# Autodesk Inventor assembly: 組合1
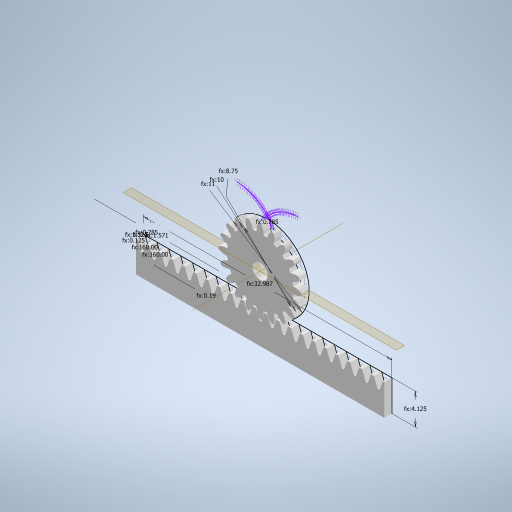
[picture p0: Inventor's stored thumbnail of the model, 512x512]
Saved by Autodesk Inventor 2024 (Build 280153000, 153)
## iProperties
Created: 2024-04-20
Part Number: 組合1
Document SubType Name: Assembly
Designer: rumse
Author: rumse
## Documents named in this file (3)
- C:\文件\機電系統實驗\Electromechanical-System-Principles\抬升機構.iam
- C:\文件\機電系統實驗\Electromechanical-System-Principles\齒條.ipt
- C:\文件\機電系統實驗\Electromechanical-System-Principles\齒輪.ipt
## Components (2 placed, 2 different names)
1. 齒輪:1 — 貼合:1, 相切:1, 貼合:2, 貼合:3, 齊平:1, 貼合:4, 旋轉/轉換:1
2. 齒條:1 — 相切:1, 貼合:2, 齊平:1, 貼合:4, 旋轉/轉換:1, 角度:1
## Relationships (8: Mate 4, Tangent 1, Flush 1, RelateRotateTranslate 1, Angle 1)
- 貼合:1 [Mate]: 齒輪:1
- 相切:1 [Tangent]: 齒輪:1 ↔ 齒條:1
- 貼合:2 [Mate]: 齒輪:1 ↔ 齒條:1
- 貼合:3 [Mate]: 齒輪:1
- 齊平:1 [Flush]: 齒輪:1 ↔ 齒條:1
- 貼合:4 [Mate]: 齒輪:1 ↔ 齒條:1
- 旋轉/轉換:1 [RelateRotateTranslate] (31.416 mm): 齒輪:1 ↔ 齒條:1
- 角度:1 [Angle] (0 deg): 齒條:1
## Named parameters: module = 0.05, teeth_number = 20, pitch_diameter = 10 mm, whole_depth = 1.125 mm, tooth_thickness = 0.7854 mm, circular_pitch = 1.5708 mm, addendum = 0.5 mm, dedendum = 0.625 mm, addendum_diameter = 11 mm, dedendum_diameter = 8.75 mm, pressure_angle = 20 deg, base_diameter = 9.39693 mm, fillet_radius = 0.19 mm, rack_tooth_number = 20, rack_length = 32.9867 mm, rack_dedendum = 0.125 mm
note: some values were not read from the file. Shown as the stored number, unit unknown: "module".
